# Autodesk Inventor assembly: Shooting Mechanism Assembly
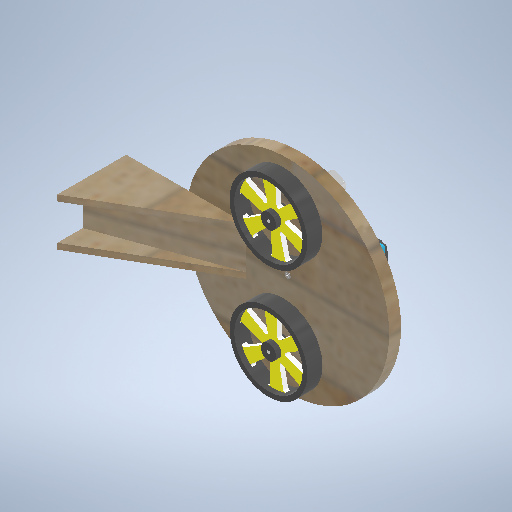
[picture p0: Inventor's stored thumbnail of the model, 512x512]
Saved by Autodesk Inventor 2025.3 (Build 293356000, 356)
## iProperties
Created: 2026-03-02
Part Number: Shooting Mechanism Assembly
Document SubType Name: Assembly
Designer: abdul
Author: abdul
## Documents named in this file (6)
- D:\Shooting Mechanism CAD\Shooting Mechanism Assembly.iam
- D:\Shooting Mechanism CAD\Base.ipt
- D:\Shooting Mechanism CAD\flywheel.ipt
- D:\Shooting Mechanism CAD\Dc Motor 3mm D Shaft.ipt
- D:\Shooting Mechanism CAD\FT7635M_Servo assembly_with T_BAR.iam
- C:\Users\abdul\OneDrive\Документы\Inventor\Content Center Files\R2025\en-US\IFI 513(1)\IFI 513 - M3x0.5 x 20(1) I.ipt
## Components (7 placed, 5 different names)
1. Base:1 — Mate:1, Mate:2, Mate:3, Mate:4, Mate:12, Mate:13, Mate:14, Mate:15
2. Dc Motor 3mm D Shaft:1 — Mate:1, Mate:4, Mate:9, Mate:11
3. Dc Motor 3mm D Shaft:2 — Mate:2, Mate:3, Mate:6, Mate:8, Mate:10
4. flywheel:2 — Mate:6, Mate:8, Mate:10
5. flywheel:3 — Mate:9, Mate:11
6. FT7635M_Servo assembly_with T_BAR:1 [sub-assembly] — Mate:12, Mate:13
7. Cross Recessed Flat Countersunk Head Machine Screw - Type I - Metric M3x0.5 x 20:1 — Mate:14, Mate:15
## Relationships (13: Mate 13)
- Mate:1: Base:1 ↔ Dc Motor 3mm D Shaft:1
- Mate:2: Base:1 ↔ Dc Motor 3mm D Shaft:2
- Mate:3: Base:1 ↔ Dc Motor 3mm D Shaft:2
- Mate:4: Base:1 ↔ Dc Motor 3mm D Shaft:1
- Mate:6: Dc Motor 3mm D Shaft:2 ↔ flywheel:2
- Mate:8: Dc Motor 3mm D Shaft:2 ↔ flywheel:2
- Mate:9: Dc Motor 3mm D Shaft:1 ↔ flywheel:3
- Mate:10: Dc Motor 3mm D Shaft:2 ↔ flywheel:2
- Mate:11: Dc Motor 3mm D Shaft:1 ↔ flywheel:3
- Mate:12: Base:1 ↔ FT7635M_Servo assembly_with T_BAR:1
- Mate:13: Base:1 ↔ FT7635M_Servo assembly_with T_BAR:1
- Mate:14: Base:1 ↔ Cross Recessed Flat Countersunk Head Machine Screw - Type I - Metric M3x0.5 x 20:1
- Mate:15: Base:1 ↔ Cross Recessed Flat Countersunk Head Machine Screw - Type I - Metric M3x0.5 x 20:1
